# Autodesk Inventor assembly: 170 Degree Hinge with Wood Screws And Cup Fixing Wood Screws
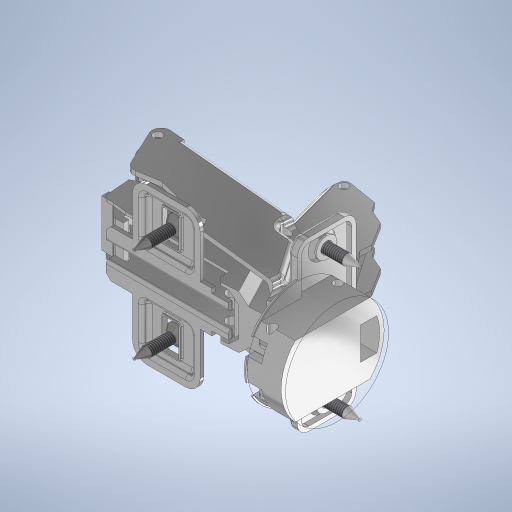
[picture p0: Inventor's stored thumbnail of the model, 512x512]
Saved by Autodesk Inventor 2024 (Build 280153000, 153)
## iProperties
Created: 2014-01-08
Part Number: 170 Degree Hinge with Wood Screws And Cup Fixing Wood Screws
Document SubType Name: Assembly
Designer: G. Kazokaitis
Author: G. Kazokaitis
## Documents named in this file (10)
- C:\W4INV 2024 Design\_LIBRARY\Hinges\170 DEGREE HINGE\170 Degree Hinge with Wood Screws And Cup Fixing Wood Screws.iam
- C:\W4INV 2024 Design\LIBRARY\Hinges\Parts\170 Degree hinge\Lever 1.ipt
- C:\W4INV 2024 Design\LIBRARY\Hinges\Parts\170 Degree hinge\Hinge case 2.ipt
- C:\W4INV 2024 Design\LIBRARY\Hinges\Parts\170 Degree hinge\Lever 2.ipt
- C:\W4INV 2024 Design\LIBRARY\Hinges\Parts\170 Degree hinge\Lever 3.ipt
- C:\W4INV 2024 Design\LIBRARY\Hinges\170 DEGREE HINGE.iam
- C:\W4INV 2024 Design\_LIBRARY\Hinges\Parts\170 Degree hinge\Mounting plate and hinge base case\170 degree Hinge with Wood Screw.ipt
- C:\W4INV 2024 Design\_LIBRARY\Hinges\Parts\170 Degree hinge\Cup for hinge\Cup for hinge with Wood screws.ipt
- C:\W4INV 2022 Design\LIBRARY\Hinges\Parts\170 Degree hinge\Cup for hinge.ipt
- C:\W4INV 2023 Design\LIBRARY\Hinges\Parts\170 Degree hinge\Mounting plate and hinge base case.ipt
## Components (6 placed, 6 different names)
1. 170 degree Hinge with Wood Screw:1 — Flush:1, Flush:2, Flush:3, Mate:1, Mate:2, Mate:5, Flush:4, Hinge Opening Angle
2. Lever 1:1 — Mate:1, Mate:2, Mate:3, Mate:4
3. Hinge case 2:1 — Mate:3, Mate:4, Mate:6, Mate:7, Mate:11
4. Lever 2:1 — Mate:5, Mate:6, Mate:7, Mate:8, Mate:9
5. Lever 3:1 — Mate:8, Mate:9, Mate:10
6. Cup for hinge with Wood screws:1 — Mate:10, Mate:11, Flush:4, Hinge Opening Angle
## Relationships (16: Mate 11, Flush 4, Angle 1)
- Flush:1: 170 degree Hinge with Wood Screw:1
- Flush:2: 170 degree Hinge with Wood Screw:1
- Flush:3: 170 degree Hinge with Wood Screw:1
- Mate:1: 170 degree Hinge with Wood Screw:1 ↔ Lever 1:1
- Mate:2 (0.25 mm): 170 degree Hinge with Wood Screw:1 ↔ Lever 1:1
- Mate:3: Lever 1:1 ↔ Hinge case 2:1
- Mate:4 (0.95 mm): Lever 1:1 ↔ Hinge case 2:1
- Mate:5: 170 degree Hinge with Wood Screw:1 ↔ Lever 2:1
- Mate:6: Hinge case 2:1 ↔ Lever 2:1
- Mate:7 (0.9 mm): Hinge case 2:1 ↔ Lever 2:1
- Mate:8: Lever 2:1 ↔ Lever 3:1
- Mate:9 (0.4 mm): Lever 2:1 ↔ Lever 3:1
- Mate:10: Lever 3:1 ↔ Cup for hinge with Wood screws:1
- Mate:11: Hinge case 2:1 ↔ Cup for hinge with Wood screws:1
- Flush:4: 170 degree Hinge with Wood Screw:1 ↔ Cup for hinge with Wood screws:1
- Hinge Opening Angle [Angle] (0 deg): 170 degree Hinge with Wood Screw:1 ↔ Cup for hinge with Wood screws:1
